# Autodesk Inventor assembly: printer
(part 2 of 3)
532. ISO 4762 M4 x 40:3 — Mate:807, Mate:809, Mate:818, Mate:826
533. ISO 4762 M4 x 40:4 — Mate:808, Mate:812, Mate:820, Mate:824
534. DIN EN ISO 7040 M4:88 — Mate:823, Mate:824
535. DIN EN ISO 7040 M4:89 — Mate:825, Mate:826
536. DIN EN ISO 7040 M4:90 — Mate:827, Mate:828
537. DIN EN ISO 7040 M4:91 — Mate:821, Mate:822
538. CSN 02 1702 B B 4,3:175 — Mate:813, Mate:818, Mate:825
539. CSN 02 1702 B B 4,3:176 — Mate:814, Mate:817, Mate:821
540. CSN 02 1702 B B 4,3:177 — Mate:815, Mate:820, Mate:823
541. CSN 02 1702 B B 4,3:178 — Mate:816, Mate:819, Mate:827
## Relationships (1028: Mate 807, Insert 155, Angle 45, Flush 17, Tangent 4)
- Mate:1: brace_left:1
- Mate:2: brace_left:1
- Flush:1: brace_left:1
- Mate:3: brace_left:1 ↔ frame:1
- Mate:4: brace_left:1 ↔ frame:1
- Mate:5: brace_left:1 ↔ frame:1
- Mate:6: frame:1 ↔ z_motor_mount:1
- Flush:2: frame:1 ↔ z_motor_mount:1
- Flush:3: frame:1 ↔ z_motor_mount:1
- Mate:7: frame:1 ↔ z_motor_mount:2
- Flush:4: frame:1 ↔ z_motor_mount:2
- Flush:5: frame:1 ↔ z_motor_mount:2
- Mate:8: z_motor_mount:1 ↔ z_rod_stopper_bottom:1
- Mate:9: z_motor_mount:1 ↔ z_rod_stopper_bottom:1
- Mate:10: z_motor_mount:1 ↔ z_rod_stopper_bottom:1
- Mate:11: z_motor_mount:2 ↔ z_rod_stopper_bottom:2
- Mate:12: z_motor_mount:2 ↔ z_rod_stopper_bottom:2
- Mate:13: z_motor_mount:2 ↔ z_rod_stopper_bottom:2
- Mate:14: z_motor_mount:1 ↔ CSN 02 1702 B B 4,3:5
- Mate:15: z_motor_mount:1 ↔ CSN 02 1702 B B 4,3:6
- Mate:16: z_motor_mount:1 ↔ CSN 02 1702 B B 4,3:5
- Mate:17: z_motor_mount:1 ↔ CSN 02 1702 B B 4,3:6
- Insert:1: CSN 02 1702 B B 4,3:5 ↔ ISO 4762 M4 x 20:4
- Insert:2: CSN 02 1702 B B 4,3:6 ↔ ISO 4762 M4 x 20:3
- Mate:18: z_rod_stopper_bottom:1 ↔ CSN 02 1702 B B 4,3:3
- Mate:19: CSN 02 1702 B B 4,3:3 ↔ ISO 4762 M4 x 20:3
- Mate:20: z_rod_stopper_bottom:1 ↔ CSN 02 1702 B B 4,3:4
- Mate:21: CSN 02 1702 B B 4,3:4 ↔ ISO 4762 M4 x 20:4
- Mate:22: z_motor_mount:2 ↔ CSN 02 1702 B B 4,3:1
- Mate:23: z_motor_mount:2 ↔ CSN 02 1702 B B 4,3:1
- Mate:24: z_motor_mount:2 ↔ CSN 02 1702 B B 4,3:8
- Mate:25: z_motor_mount:2 ↔ CSN 02 1702 B B 4,3:8
- Insert:3: CSN 02 1702 B B 4,3:8 ↔ ISO 4762 M4 x 20:2
- Insert:4: CSN 02 1702 B B 4,3:1 ↔ ISO 4762 M4 x 20:1
- Mate:26: z_rod_stopper_bottom:2 ↔ CSN 02 1702 B B 4,3:2
- Mate:27: CSN 02 1702 B B 4,3:2 ↔ ISO 4762 M4 x 20:2
- Mate:28: z_rod_stopper_bottom:2 ↔ CSN 02 1702 B B 4,3:7
- Mate:29: CSN 02 1702 B B 4,3:7 ↔ ISO 4762 M4 x 20:1
- Mate:30: CSN 02 1702 B B 4,3:3 ↔ DIN EN ISO 7040 M4:4
- Mate:31: ISO 4762 M4 x 20:3 ↔ DIN EN ISO 7040 M4:4
- Mate:32: CSN 02 1702 B B 4,3:4 ↔ DIN EN ISO 7040 M4:3
- Mate:33: ISO 4762 M4 x 20:4 ↔ DIN EN ISO 7040 M4:3
- Mate:34: CSN 02 1702 B B 4,3:2 ↔ DIN EN ISO 7040 M4:2
- Mate:35: ISO 4762 M4 x 20:2 ↔ DIN EN ISO 7040 M4:2
- Mate:36: CSN 02 1702 B B 4,3:7 ↔ DIN EN ISO 7040 M4:1
- Mate:37: ISO 4762 M4 x 20:1 ↔ DIN EN ISO 7040 M4:1
- Mate:38: z_rod_stopper_bottom:1 ↔ NEMA 17:1
- Mate:39: z_rod_stopper_bottom:1 ↔ NEMA 17:1
- Mate:40: z_rod_stopper_bottom:1 ↔ NEMA 17:1
- Mate:41: z_rod_stopper_bottom:2 ↔ NEMA 17:2
- Mate:42: z_rod_stopper_bottom:2 ↔ NEMA 17:2
- Mate:43: z_rod_stopper_bottom:2 ↔ NEMA 17:2
- Mate:44: z_motor_mount:1 ↔ CSN 02 1702 B B 3,2:8
- Mate:45: z_motor_mount:1 ↔ CSN 02 1702 B B 3,2:1
- Mate:46: z_motor_mount:1 ↔ CSN 02 1702 B B 3,2:6
- Mate:47: z_motor_mount:1 ↔ CSN 02 1702 B B 3,2:7
- Mate:48: z_motor_mount:2 ↔ CSN 02 1702 B B 3,2:2
- Mate:49: z_motor_mount:2 ↔ CSN 02 1702 B B 3,2:3
- Mate:50: z_motor_mount:2 ↔ CSN 02 1702 B B 3,2:4
- Mate:51: z_motor_mount:2 ↔ CSN 02 1702 B B 3,2:5
- Mate:52: z_motor_mount:1 ↔ CSN 02 1702 B B 3,2:8
- Mate:53: z_motor_mount:1 ↔ CSN 02 1702 B B 3,2:1
- Mate:54: z_motor_mount:1 ↔ CSN 02 1702 B B 3,2:7
- Mate:55: z_motor_mount:1 ↔ CSN 02 1702 B B 3,2:6
- Mate:56: z_motor_mount:2 ↔ CSN 02 1702 B B 3,2:5
- Mate:57: z_motor_mount:2 ↔ CSN 02 1702 B B 3,2:2
- Mate:58: z_motor_mount:2 ↔ CSN 02 1702 B B 3,2:4
- Mate:59: z_motor_mount:2 ↔ CSN 02 1702 B B 3,2:3
- Insert:5: CSN 02 1702 B B 3,2:7 ↔ ISO 4762 M3 x 20:8
- Insert:6: CSN 02 1702 B B 3,2:8 ↔ ISO 4762 M3 x 20:7
- Insert:7: CSN 02 1702 B B 3,2:6 ↔ ISO 4762 M3 x 20:6
- Insert:8: CSN 02 1702 B B 3,2:1 ↔ ISO 4762 M3 x 20:5
- Insert:9: CSN 02 1702 B B 3,2:5 ↔ ISO 4762 M3 x 20:4
- Insert:10: CSN 02 1702 B B 3,2:2 ↔ ISO 4762 M3 x 20:3
- Insert:11: CSN 02 1702 B B 3,2:3 ↔ ISO 4762 M3 x 20:2
- Insert:12: CSN 02 1702 B B 3,2:4 ↔ ISO 4762 M3 x 20:1
- Insert:13: z_motor_mount:1 ↔ z_axis_rod:2
- Insert:14: z_motor_mount:2 ↔ z_axis_rod:1
- Mate:60: z_motor_mount:2 ↔ z_motor_brace:1
- Mate:61: z_motor_mount:2 ↔ z_motor_brace:1
- Mate:62: z_motor_mount:2 ↔ z_motor_brace:1
- Mate:63: z_motor_mount:1 ↔ z_motor_brace:2
- Mate:64: z_motor_mount:1 ↔ z_motor_brace:2
- Mate:65: z_motor_mount:1 ↔ z_motor_brace:2
- Mate:66: NEMA 17:1 ↔ z_threaded_rod:1
- Mate:67: NEMA 17:1 ↔ z_threaded_rod:1
- Mate:68: NEMA 17:2 ↔ z_threaded_rod:2
- Mate:69: NEMA 17:2 ↔ z_threaded_rod:2
- Mate:70: frame:1 ↔ frame_brace_top:1
- Mate:71: brace_left:1 ↔ frame_brace_top:1
- Mate:72: frame:1 ↔ frame_brace_top:1
- Mate:73: brace_left:1 ↔ front:1
- Flush:6: brace_left:1 ↔ front:1
- Flush:7 (-3 mm): brace_left:1 ↔ front:1
- Mate:74: frame:1 ↔ z_axis_top:1
- Mate:75: frame:1 ↔ z_axis_top:1
- Mate:76: frame:1 ↔ z_axis_top:1
- Mate:77: frame:1 ↔ z_axis_top:2
- Mate:78: frame:1 ↔ z_axis_top:2
- Mate:79: frame:1 ↔ z_axis_top:2
- Mate:80: brace_left:1 ↔ bottom:1
- Mate:81: front:1 ↔ bottom:1
- Flush:8 (3 mm): brace_left:1 ↔ bottom:1
- Mate:84: frame:1 ↔ wiring_brace:1
- Flush:9: frame:1 ↔ wiring_brace:1
- Mate:85: brace_left:1 ↔ wiring_brace:1
- Mate:86: frame:1 ↔ wiring_brace:2
- Flush:10: frame:1 ↔ wiring_brace:2
- Mate:87: frame:1 ↔ wiring_brace:2
- Mate:88: frame:1 ↔ brace_right:1
- Mate:89: bottom:1 ↔ brace_right:1
- Flush:11 (-3 mm): bottom:1 ↔ brace_right:1
- Mate:90: brace_right:1 ↔ back:1
- Flush:12 (-3 mm): brace_right:1 ↔ back:1
- Flush:13 (-3 mm): bottom:1 ↔ back:1
- Insert:15: front:1 ↔ y_axis_rod:2
- Insert:16: front:1 ↔ y_axis_rod:1
- Mate:91: front:1 ↔ CSN 02 1702 B B 4,3:18
- Mate:92: front:1 ↔ CSN 02 1702 B B 4,3:17
- Mate:93: front:1 ↔ CSN 02 1702 B B 4,3:16
- Mate:94: front:1 ↔ CSN 02 1702 B B 4,3:13
- Mate:95: front:1 ↔ CSN 02 1702 B B 4,3:14
- Mate:96: front:1 ↔ CSN 02 1702 B B 4,3:15
- Mate:97: front:1 ↔ CSN 02 1702 B B 4,3:9
- Mate:98: front:1 ↔ CSN 02 1702 B B 4,3:10
- Mate:99: front:1 ↔ CSN 02 1702 B B 4,3:11
- Mate:100: front:1 ↔ CSN 02 1702 B B 4,3:22
- Mate:101: front:1 ↔ CSN 02 1702 B B 4,3:18
- Mate:102: front:1 ↔ CSN 02 1702 B B 4,3:17
- Mate:103: front:1 ↔ CSN 02 1702 B B 4,3:16
- Mate:104: front:1 ↔ CSN 02 1702 B B 4,3:13
- Mate:105: front:1 ↔ CSN 02 1702 B B 4,3:14
- Mate:106: front:1 ↔ CSN 02 1702 B B 4,3:15
- Mate:107: front:1 ↔ CSN 02 1702 B B 4,3:9
- Mate:108: front:1 ↔ CSN 02 1702 B B 4,3:10
- Mate:109: front:1 ↔ CSN 02 1702 B B 4,3:11
- Mate:110: front:1 ↔ CSN 02 1702 B B 4,3:22
- Insert:17: CSN 02 1702 B B 4,3:18 ↔ ISO 4762 M4 x 20:5
- Insert:18: CSN 02 1702 B B 4,3:17 ↔ ISO 4762 M4 x 20:6
- Insert:19: CSN 02 1702 B B 4,3:16 ↔ ISO 4762 M4 x 20:7
- Insert:20: CSN 02 1702 B B 4,3:13 ↔ ISO 4762 M4 x 20:8
- Insert:21: CSN 02 1702 B B 4,3:14 ↔ ISO 4762 M4 x 20:9
- Insert:22: CSN 02 1702 B B 4,3:15 ↔ ISO 4762 M4 x 20:10
- Insert:23: CSN 02 1702 B B 4,3:9 ↔ ISO 4762 M4 x 20:11
- Insert:24: CSN 02 1702 B B 4,3:10 ↔ ISO 4762 M4 x 20:12
- Insert:25: CSN 02 1702 B B 4,3:11 ↔ ISO 4762 M4 x 20:13
- Insert:26: CSN 02 1702 B B 4,3:22 ↔ ISO 4762 M4 x 20:14
- Mate:111: brace_left:1 ↔ CSN 02 1702 B B 4,3:28
- Mate:112: CSN 02 1702 B B 4,3:28 ↔ ISO 4762 M4 x 20:5
- Mate:113: brace_left:1 ↔ CSN 02 1702 B B 4,3:25
- Mate:114: CSN 02 1702 B B 4,3:25 ↔ ISO 4762 M4 x 20:6
- Mate:115: brace_left:1 ↔ CSN 02 1702 B B 4,3:21
- Mate:116: CSN 02 1702 B B 4,3:21 ↔ ISO 4762 M4 x 20:7
- Mate:117: bottom:1 ↔ CSN 02 1702 B B 4,3:20
- Mate:118: CSN 02 1702 B B 4,3:20 ↔ ISO 4762 M4 x 20:8
- Mate:119: bottom:1 ↔ CSN 02 1702 B B 4,3:27
- Mate:120: CSN 02 1702 B B 4,3:27 ↔ ISO 4762 M4 x 20:9
- Mate:121: bottom:1 ↔ CSN 02 1702 B B 4,3:24
- Mate:122: CSN 02 1702 B B 4,3:24 ↔ ISO 4762 M4 x 20:10
- Mate:123: bottom:1 ↔ CSN 02 1702 B B 4,3:26
- Mate:124: CSN 02 1702 B B 4,3:26 ↔ ISO 4762 M4 x 20:11
- Mate:125: brace_right:1 ↔ CSN 02 1702 B B 4,3:23
- Mate:126: CSN 02 1702 B B 4,3:23 ↔ ISO 4762 M4 x 20:14
- Mate:127: brace_right:1 ↔ CSN 02 1702 B B 4,3:19
- Mate:128: CSN 02 1702 B B 4,3:19 ↔ ISO 4762 M4 x 20:13
- Mate:129: brace_right:1 ↔ CSN 02 1702 B B 4,3:12
- Mate:130: CSN 02 1702 B B 4,3:12 ↔ ISO 4762 M4 x 20:12
- Mate:131: CSN 02 1702 B B 4,3:28 ↔ DIN EN ISO 7040 M4:5
- Mate:132: ISO 4762 M4 x 20:5 ↔ DIN EN ISO 7040 M4:5
- Mate:133: CSN 02 1702 B B 4,3:25 ↔ DIN EN ISO 7040 M4:12
- Mate:134: ISO 4762 M4 x 20:6 ↔ DIN EN ISO 7040 M4:12
- Mate:135: CSN 02 1702 B B 4,3:21 ↔ DIN EN ISO 7040 M4:9
- Mate:136: ISO 4762 M4 x 20:7 ↔ DIN EN ISO 7040 M4:9
- Mate:137: CSN 02 1702 B B 4,3:20 ↔ DIN EN ISO 7040 M4:13
- Mate:138: ISO 4762 M4 x 20:8 ↔ DIN EN ISO 7040 M4:13
- Mate:139: CSN 02 1702 B B 4,3:27 ↔ DIN EN ISO 7040 M4:14
- Mate:140: ISO 4762 M4 x 20:9 ↔ DIN EN ISO 7040 M4:14
- Mate:141: CSN 02 1702 B B 4,3:24 ↔ DIN EN ISO 7040 M4:6
- Mate:142: ISO 4762 M4 x 20:10 ↔ DIN EN ISO 7040 M4:6
- Mate:143: CSN 02 1702 B B 4,3:26 ↔ DIN EN ISO 7040 M4:7
- Mate:144: ISO 4762 M4 x 20:11 ↔ DIN EN ISO 7040 M4:7
- Mate:145: CSN 02 1702 B B 4,3:23 ↔ DIN EN ISO 7040 M4:10
- Mate:146: ISO 4762 M4 x 20:14 ↔ DIN EN ISO 7040 M4:10
- Mate:147: CSN 02 1702 B B 4,3:19 ↔ DIN EN ISO 7040 M4:8
- Mate:148: ISO 4762 M4 x 20:13 ↔ DIN EN ISO 7040 M4:8
- Mate:149: CSN 02 1702 B B 4,3:12 ↔ DIN EN ISO 7040 M4:11
- Mate:150: ISO 4762 M4 x 20:12 ↔ DIN EN ISO 7040 M4:11
- Mate:151: back:1 ↔ CSN 02 1702 B B 4,3:29
- Mate:152: back:1 ↔ CSN 02 1702 B B 4,3:30
- Mate:153: back:1 ↔ CSN 02 1702 B B 4,3:32
- Mate:154: back:1 ↔ CSN 02 1702 B B 4,3:33
- Mate:155: back:1 ↔ CSN 02 1702 B B 4,3:35
- Mate:156: back:1 ↔ CSN 02 1702 B B 4,3:36
- Mate:157: back:1 ↔ CSN 02 1702 B B 4,3:37
- Mate:158: back:1 ↔ CSN 02 1702 B B 4,3:38
- Mate:159: back:1 ↔ CSN 02 1702 B B 4,3:34
- Mate:160: back:1 ↔ CSN 02 1702 B B 4,3:31
- Mate:161: back:1 ↔ CSN 02 1702 B B 4,3:31
- Mate:162: back:1 ↔ CSN 02 1702 B B 4,3:34
- Mate:163: back:1 ↔ CSN 02 1702 B B 4,3:38
- Mate:164: back:1 ↔ CSN 02 1702 B B 4,3:37
- Mate:165: back:1 ↔ CSN 02 1702 B B 4,3:36
- Mate:166: back:1 ↔ CSN 02 1702 B B 4,3:35
- Mate:167: back:1 ↔ CSN 02 1702 B B 4,3:33
- Mate:168: back:1 ↔ CSN 02 1702 B B 4,3:29
- Mate:169: back:1 ↔ CSN 02 1702 B B 4,3:30
- Mate:170: back:1 ↔ CSN 02 1702 B B 4,3:32
- Insert:27: CSN 02 1702 B B 4,3:32 ↔ ISO 4762 M4 x 20:15
- Insert:28: CSN 02 1702 B B 4,3:30 ↔ ISO 4762 M4 x 20:16
- Insert:29: CSN 02 1702 B B 4,3:29 ↔ ISO 4762 M4 x 20:17
- Insert:30: CSN 02 1702 B B 4,3:33 ↔ ISO 4762 M4 x 20:18
- Insert:31: CSN 02 1702 B B 4,3:35 ↔ ISO 4762 M4 x 20:19
- Insert:32: CSN 02 1702 B B 4,3:36 ↔ ISO 4762 M4 x 20:20
- Insert:33: CSN 02 1702 B B 4,3:37 ↔ ISO 4762 M4 x 20:21
- Insert:34: CSN 02 1702 B B 4,3:38 ↔ ISO 4762 M4 x 20:22
- Insert:35: CSN 02 1702 B B 4,3:34 ↔ ISO 4762 M4 x 20:23
- Insert:36: CSN 02 1702 B B 4,3:31 ↔ ISO 4762 M4 x 20:24
- Mate:171: brace_right:1 ↔ CSN 02 1702 B B 4,3:39
- Mate:172: CSN 02 1702 B B 4,3:39 ↔ ISO 4762 M4 x 20:24
- Mate:173: brace_right:1 ↔ CSN 02 1702 B B 4,3:41
- Mate:174: CSN 02 1702 B B 4,3:41 ↔ ISO 4762 M4 x 20:23
- Mate:175: brace_right:1 ↔ CSN 02 1702 B B 4,3:40
- Mate:176: CSN 02 1702 B B 4,3:40 ↔ ISO 4762 M4 x 20:22
- Mate:177: brace_left:1 ↔ CSN 02 1702 B B 4,3:42
- Mate:178: CSN 02 1702 B B 4,3:42 ↔ ISO 4762 M4 x 20:15
- Mate:179: brace_left:1 ↔ CSN 02 1702 B B 4,3:45
- Mate:180: CSN 02 1702 B B 4,3:45 ↔ ISO 4762 M4 x 20:16
- Mate:181: brace_left:1 ↔ CSN 02 1702 B B 4,3:43
- Mate:182: CSN 02 1702 B B 4,3:43 ↔ ISO 4762 M4 x 20:17
- Mate:183: bottom:1 ↔ CSN 02 1702 B B 4,3:46
- Mate:184: CSN 02 1702 B B 4,3:46 ↔ ISO 4762 M4 x 20:18
- Mate:185: bottom:1 ↔ CSN 02 1702 B B 4,3:47
- Mate:186: CSN 02 1702 B B 4,3:47 ↔ ISO 4762 M4 x 20:19
- Mate:187: bottom:1 ↔ CSN 02 1702 B B 4,3:44
- Mate:188: CSN 02 1702 B B 4,3:44 ↔ ISO 4762 M4 x 20:20
- Mate:189: bottom:1 ↔ CSN 02 1702 B B 4,3:48
- Mate:190: CSN 02 1702 B B 4,3:48 ↔ ISO 4762 M4 x 20:21
- Mate:191: CSN 02 1702 B B 4,3:42 ↔ DIN EN ISO 7040 M4:17
- Mate:192: ISO 4762 M4 x 20:15 ↔ DIN EN ISO 7040 M4:17
- Mate:193: CSN 02 1702 B B 4,3:45 ↔ DIN EN ISO 7040 M4:15
- Mate:194: ISO 4762 M4 x 20:16 ↔ DIN EN ISO 7040 M4:15
- Mate:195: CSN 02 1702 B B 4,3:43 ↔ DIN EN ISO 7040 M4:22
- Mate:196: ISO 4762 M4 x 20:17 ↔ DIN EN ISO 7040 M4:22
- Mate:197: CSN 02 1702 B B 4,3:46 ↔ DIN EN ISO 7040 M4:23
- Mate:198: ISO 4762 M4 x 20:18 ↔ DIN EN ISO 7040 M4:23
- Mate:199: CSN 02 1702 B B 4,3:47 ↔ DIN EN ISO 7040 M4:24
- Mate:200: ISO 4762 M4 x 20:19 ↔ DIN EN ISO 7040 M4:24
- Mate:201: CSN 02 1702 B B 4,3:44 ↔ DIN EN ISO 7040 M4:18
- Mate:202: ISO 4762 M4 x 20:20 ↔ DIN EN ISO 7040 M4:18
- Mate:203: CSN 02 1702 B B 4,3:48 ↔ DIN EN ISO 7040 M4:21
- Mate:204: ISO 4762 M4 x 20:21 ↔ DIN EN ISO 7040 M4:21
- Mate:205: CSN 02 1702 B B 4,3:39 ↔ DIN EN ISO 7040 M4:20
- Mate:206: ISO 4762 M4 x 20:24 ↔ DIN EN ISO 7040 M4:20
- Mate:207: CSN 02 1702 B B 4,3:41 ↔ DIN EN ISO 7040 M4:16
- Mate:208: ISO 4762 M4 x 20:23 ↔ DIN EN ISO 7040 M4:16
- Mate:209: CSN 02 1702 B B 4,3:40 ↔ DIN EN ISO 7040 M4:19
- Mate:210: ISO 4762 M4 x 20:22 ↔ DIN EN ISO 7040 M4:19
- Mate:211: frame:1 ↔ CSN 02 1702 B B 4,3:49
- Mate:212: frame:1 ↔ CSN 02 1702 B B 4,3:59
- Mate:213: frame:1 ↔ CSN 02 1702 B B 4,3:50
- Mate:214: frame:1 ↔ CSN 02 1702 B B 4,3:51
- Mate:215: frame:1 ↔ CSN 02 1702 B B 4,3:52
- Mate:216: frame:1 ↔ CSN 02 1702 B B 4,3:53
- Mate:217: frame:1 ↔ CSN 02 1702 B B 4,3:54
- Mate:218: frame:1 ↔ CSN 02 1702 B B 4,3:55
- Mate:219: frame:1 ↔ CSN 02 1702 B B 4,3:56
- Mate:220: frame:1 ↔ CSN 02 1702 B B 4,3:57
- Mate:221: frame:1 ↔ CSN 02 1702 B B 4,3:53
- Mate:222: frame:1 ↔ CSN 02 1702 B B 4,3:54
- Mate:223: frame:1 ↔ CSN 02 1702 B B 4,3:55
- Mate:224: frame:1 ↔ CSN 02 1702 B B 4,3:56
- Mate:225: frame:1 ↔ CSN 02 1702 B B 4,3:57
- Mate:226: frame:1 ↔ CSN 02 1702 B B 4,3:49
- Mate:227: frame:1 ↔ CSN 02 1702 B B 4,3:59
- Mate:228: frame:1 ↔ CSN 02 1702 B B 4,3:50
- Mate:229: frame:1 ↔ CSN 02 1702 B B 4,3:51
- Mate:230: frame:1 ↔ CSN 02 1702 B B 4,3:52
- Insert:37: CSN 02 1702 B B 4,3:49 ↔ ISO 4762 M4 x 20:25
- Insert:38: CSN 02 1702 B B 4,3:59 ↔ ISO 4762 M4 x 20:26
- Insert:39: CSN 02 1702 B B 4,3:50 ↔ ISO 4762 M4 x 20:27
- Insert:40: CSN 02 1702 B B 4,3:51 ↔ ISO 4762 M4 x 20:28
- Insert:41: CSN 02 1702 B B 4,3:52 ↔ ISO 4762 M4 x 20:29
- Insert:42: CSN 02 1702 B B 4,3:53 ↔ ISO 4762 M4 x 20:30
- Insert:43: CSN 02 1702 B B 4,3:54 ↔ ISO 4762 M4 x 20:31
- Insert:44: CSN 02 1702 B B 4,3:55 ↔ ISO 4762 M4 x 20:32
- Insert:45: CSN 02 1702 B B 4,3:56 ↔ ISO 4762 M4 x 20:33
- Insert:46: CSN 02 1702 B B 4,3:57 ↔ ISO 4762 M4 x 20:34
- Mate:231: brace_right:1 ↔ CSN 02 1702 B B 4,3:60
- Mate:232: CSN 02 1702 B B 4,3:60 ↔ ISO 4762 M4 x 20:25
- Mate:233: brace_right:1 ↔ CSN 02 1702 B B 4,3:61
- Mate:234: CSN 02 1702 B B 4,3:61 ↔ ISO 4762 M4 x 20:26
- Mate:235: brace_right:1 ↔ CSN 02 1702 B B 4,3:62
- Mate:236: CSN 02 1702 B B 4,3:62 ↔ ISO 4762 M4 x 20:27
- Mate:237: brace_right:1 ↔ CSN 02 1702 B B 4,3:63
- Mate:238: CSN 02 1702 B B 4,3:63 ↔ ISO 4762 M4 x 20:28
- Mate:239: brace_right:1 ↔ CSN 02 1702 B B 4,3:64
- Mate:240: CSN 02 1702 B B 4,3:64 ↔ ISO 4762 M4 x 20:29
- Mate:241: brace_left:1 ↔ CSN 02 1702 B B 4,3:65
- Mate:242: CSN 02 1702 B B 4,3:65 ↔ ISO 4762 M4 x 20:30
- Mate:243: brace_left:1 ↔ CSN 02 1702 B B 4,3:66
- Mate:244: CSN 02 1702 B B 4,3:66 ↔ ISO 4762 M4 x 20:31
- Mate:245: brace_left:1 ↔ CSN 02 1702 B B 4,3:67
- Mate:246: CSN 02 1702 B B 4,3:67 ↔ ISO 4762 M4 x 20:32
- Mate:247: brace_left:1 ↔ CSN 02 1702 B B 4,3:58
- Mate:248: CSN 02 1702 B B 4,3:58 ↔ ISO 4762 M4 x 20:33
- Mate:249: brace_left:1 ↔ CSN 02 1702 B B 4,3:68
- Mate:250: CSN 02 1702 B B 4,3:68 ↔ ISO 4762 M4 x 20:34
- Mate:251: CSN 02 1702 B B 4,3:60 ↔ DIN EN ISO 7040 M4:25
- Mate:252: ISO 4762 M4 x 20:25 ↔ DIN EN ISO 7040 M4:25
- Mate:253: CSN 02 1702 B B 4,3:61 ↔ DIN EN ISO 7040 M4:26
- Mate:254: ISO 4762 M4 x 20:26 ↔ DIN EN ISO 7040 M4:26
- Mate:255: CSN 02 1702 B B 4,3:62 ↔ DIN EN ISO 7040 M4:27
- Mate:256: ISO 4762 M4 x 20:27 ↔ DIN EN ISO 7040 M4:27
- Mate:257: CSN 02 1702 B B 4,3:63 ↔ DIN EN ISO 7040 M4:34
- Mate:258: ISO 4762 M4 x 20:28 ↔ DIN EN ISO 7040 M4:34
- Mate:259: CSN 02 1702 B B 4,3:64 ↔ DIN EN ISO 7040 M4:33
- Mate:260: ISO 4762 M4 x 20:29 ↔ DIN EN ISO 7040 M4:33
- Mate:261: CSN 02 1702 B B 4,3:65 ↔ DIN EN ISO 7040 M4:28
- Mate:262: ISO 4762 M4 x 20:30 ↔ DIN EN ISO 7040 M4:28
- Mate:263: CSN 02 1702 B B 4,3:66 ↔ DIN EN ISO 7040 M4:29
- Mate:264: ISO 4762 M4 x 20:31 ↔ DIN EN ISO 7040 M4:29
- Mate:265: CSN 02 1702 B B 4,3:67 ↔ DIN EN ISO 7040 M4:32
- Mate:266: ISO 4762 M4 x 20:32 ↔ DIN EN ISO 7040 M4:32
- Mate:267: CSN 02 1702 B B 4,3:58 ↔ DIN EN ISO 7040 M4:30
- Mate:268: ISO 4762 M4 x 20:33 ↔ DIN EN ISO 7040 M4:30
- Mate:269: CSN 02 1702 B B 4,3:68 ↔ DIN EN ISO 7040 M4:31
- Mate:270: ISO 4762 M4 x 20:34 ↔ DIN EN ISO 7040 M4:31
- Mate:271: brace_right:1 ↔ CSN 02 1702 B B 4,3:69
- Mate:272: brace_right:1 ↔ CSN 02 1702 B B 4,3:70
- Mate:273: brace_right:1 ↔ CSN 02 1702 B B 4,3:71
- Mate:274: brace_right:1 ↔ CSN 02 1702 B B 4,3:72
- Mate:275: brace_right:1 ↔ CSN 02 1702 B B 4,3:73
- Mate:276: brace_left:1 ↔ CSN 02 1702 B B 4,3:74
- Mate:277: brace_left:1 ↔ CSN 02 1702 B B 4,3:75
- Mate:278: brace_left:1 ↔ CSN 02 1702 B B 4,3:76
- Mate:279: brace_left:1 ↔ CSN 02 1702 B B 4,3:77
- Mate:280: brace_left:1 ↔ CSN 02 1702 B B 4,3:78
- Mate:281: brace_left:1 ↔ CSN 02 1702 B B 4,3:74
- Mate:282: brace_left:1 ↔ CSN 02 1702 B B 4,3:75
- Mate:283: brace_left:1 ↔ CSN 02 1702 B B 4,3:76
- Mate:284: brace_left:1 ↔ CSN 02 1702 B B 4,3:77
- Mate:285: brace_left:1 ↔ CSN 02 1702 B B 4,3:78
- Mate:286: brace_right:1 ↔ CSN 02 1702 B B 4,3:73
- Mate:287: brace_right:1 ↔ CSN 02 1702 B B 4,3:72
- Mate:288: brace_right:1 ↔ CSN 02 1702 B B 4,3:71
- Mate:289: brace_right:1 ↔ CSN 02 1702 B B 4,3:70
- Mate:290: brace_right:1 ↔ CSN 02 1702 B B 4,3:69
- Insert:47: CSN 02 1702 B B 4,3:73 ↔ ISO 4762 M4 x 20:44
- Insert:48: CSN 02 1702 B B 4,3:72 ↔ ISO 4762 M4 x 20:43
- Insert:49: CSN 02 1702 B B 4,3:71 ↔ ISO 4762 M4 x 20:42
- Insert:50: CSN 02 1702 B B 4,3:70 ↔ ISO 4762 M4 x 20:41
- Insert:51: CSN 02 1702 B B 4,3:69 ↔ ISO 4762 M4 x 20:40
- Insert:52: CSN 02 1702 B B 4,3:78 ↔ ISO 4762 M4 x 20:39
- Insert:53: CSN 02 1702 B B 4,3:77 ↔ ISO 4762 M4 x 20:38
- Insert:54: CSN 02 1702 B B 4,3:76 ↔ ISO 4762 M4 x 20:37
- Insert:55: CSN 02 1702 B B 4,3:75 ↔ ISO 4762 M4 x 20:36
- Insert:56: CSN 02 1702 B B 4,3:74 ↔ ISO 4762 M4 x 20:35
- Mate:291: bottom:1 ↔ CSN 02 1702 B B 4,3:88
- Mate:292: CSN 02 1702 B B 4,3:88 ↔ ISO 4762 M4 x 20:39
- Mate:293: bottom:1 ↔ CSN 02 1702 B B 4,3:87
- Mate:294: CSN 02 1702 B B 4,3:87 ↔ ISO 4762 M4 x 20:38
- Mate:295: bottom:1 ↔ CSN 02 1702 B B 4,3:86
- Mate:296: CSN 02 1702 B B 4,3:86 ↔ ISO 4762 M4 x 20:37
- Mate:297: bottom:1 ↔ CSN 02 1702 B B 4,3:85
- Mate:298: CSN 02 1702 B B 4,3:85 ↔ ISO 4762 M4 x 20:36
- Mate:299: bottom:1 ↔ CSN 02 1702 B B 4,3:84
- Mate:300: CSN 02 1702 B B 4,3:84 ↔ ISO 4762 M4 x 20:35
- Mate:301: bottom:1 ↔ CSN 02 1702 B B 4,3:83
- Mate:302: CSN 02 1702 B B 4,3:83 ↔ ISO 4762 M4 x 20:40
- Mate:303: bottom:1 ↔ CSN 02 1702 B B 4,3:79
- Mate:304: CSN 02 1702 B B 4,3:79 ↔ ISO 4762 M4 x 20:41
- Mate:305: bottom:1 ↔ CSN 02 1702 B B 4,3:80
- Mate:306: CSN 02 1702 B B 4,3:80 ↔ ISO 4762 M4 x 20:42
- Mate:307: bottom:1 ↔ CSN 02 1702 B B 4,3:81
- Mate:308: CSN 02 1702 B B 4,3:81 ↔ ISO 4762 M4 x 20:43
- Mate:309: bottom:1 ↔ CSN 02 1702 B B 4,3:82
- Mate:310: CSN 02 1702 B B 4,3:82 ↔ ISO 4762 M4 x 20:44
- Mate:311: CSN 02 1702 B B 4,3:82 ↔ DIN EN ISO 7040 M4:41
- Mate:312: ISO 4762 M4 x 20:44 ↔ DIN EN ISO 7040 M4:41
- Mate:313: CSN 02 1702 B B 4,3:81 ↔ DIN EN ISO 7040 M4:40
- Mate:314: ISO 4762 M4 x 20:43 ↔ DIN EN ISO 7040 M4:40
- Mate:315: CSN 02 1702 B B 4,3:80 ↔ DIN EN ISO 7040 M4:39
- Mate:316: ISO 4762 M4 x 20:42 ↔ DIN EN ISO 7040 M4:39
- Mate:317: CSN 02 1702 B B 4,3:79 ↔ DIN EN ISO 7040 M4:38
- Mate:318: ISO 4762 M4 x 20:41 ↔ DIN EN ISO 7040 M4:38
- Mate:319: CSN 02 1702 B B 4,3:83 ↔ DIN EN ISO 7040 M4:42
- Mate:320: ISO 4762 M4 x 20:40 ↔ DIN EN ISO 7040 M4:42
- Mate:321: CSN 02 1702 B B 4,3:88 ↔ DIN EN ISO 7040 M4:37
- Mate:322: ISO 4762 M4 x 20:39 ↔ DIN EN ISO 7040 M4:37
- Mate:323: CSN 02 1702 B B 4,3:87 ↔ DIN EN ISO 7040 M4:43
- Mate:324: ISO 4762 M4 x 20:38 ↔ DIN EN ISO 7040 M4:43
- Mate:325: CSN 02 1702 B B 4,3:85 ↔ DIN EN ISO 7040 M4:44
- Mate:326: ISO 4762 M4 x 20:36 ↔ DIN EN ISO 7040 M4:44
- Mate:327: CSN 02 1702 B B 4,3:86 ↔ DIN EN ISO 7040 M4:36
- Mate:328: ISO 4762 M4 x 20:37 ↔ DIN EN ISO 7040 M4:36
- Mate:329: CSN 02 1702 B B 4,3:84 ↔ DIN EN ISO 7040 M4:35
- Mate:330: ISO 4762 M4 x 20:35 ↔ DIN EN ISO 7040 M4:35
- Mate:331: z_motor_mount:2 ↔ CSN 02 1702 B B 4,3:98
- Mate:332: z_motor_mount:2 ↔ CSN 02 1702 B B 4,3:97
- Mate:333: frame:1 ↔ CSN 02 1702 B B 4,3:96
- Mate:334: frame:1 ↔ CSN 02 1702 B B 4,3:95
- Mate:335: frame:1 ↔ CSN 02 1702 B B 4,3:94
- Mate:336: frame:1 ↔ CSN 02 1702 B B 4,3:93
- Mate:337: frame:1 ↔ CSN 02 1702 B B 4,3:92
- Mate:338: frame:1 ↔ CSN 02 1702 B B 4,3:91
- Mate:339: z_motor_mount:1 ↔ CSN 02 1702 B B 4,3:90
- Mate:340: z_motor_mount:1 ↔ CSN 02 1702 B B 4,3:89
- Mate:341: z_motor_mount:1 ↔ CSN 02 1702 B B 4,3:89
- Mate:342: z_motor_mount:1 ↔ CSN 02 1702 B B 4,3:90
- Mate:343: frame:1 ↔ CSN 02 1702 B B 4,3:93
- Mate:344: frame:1 ↔ CSN 02 1702 B B 4,3:92
- Mate:345: frame:1 ↔ CSN 02 1702 B B 4,3:91
- Mate:346: frame:1 ↔ CSN 02 1702 B B 4,3:96
- Mate:347: frame:1 ↔ CSN 02 1702 B B 4,3:95
- Mate:348: frame:1 ↔ CSN 02 1702 B B 4,3:94
- Mate:349: z_motor_mount:2 ↔ CSN 02 1702 B B 4,3:97
- Mate:350: z_motor_mount:2 ↔ CSN 02 1702 B B 4,3:98
- Insert:57: CSN 02 1702 B B 4,3:97 ↔ ISO 4762 M4 x 20:54
- Insert:58: CSN 02 1702 B B 4,3:98 ↔ ISO 4762 M4 x 20:53
- Insert:59: CSN 02 1702 B B 4,3:95 ↔ ISO 4762 M4 x 20:52
- Insert:60: CSN 02 1702 B B 4,3:96 ↔ ISO 4762 M4 x 20:51
- Insert:61: CSN 02 1702 B B 4,3:94 ↔ ISO 4762 M4 x 20:50
- Insert:62: CSN 02 1702 B B 4,3:93 ↔ ISO 4762 M4 x 20:49
- Insert:63: CSN 02 1702 B B 4,3:92 ↔ ISO 4762 M4 x 20:48
- Insert:64: CSN 02 1702 B B 4,3:91 ↔ ISO 4762 M4 x 20:45
- Insert:65: CSN 02 1702 B B 4,3:89 ↔ ISO 4762 M4 x 20:46
- Insert:66: CSN 02 1702 B B 4,3:90 ↔ ISO 4762 M4 x 20:47
- Mate:351: z_motor_brace:1 ↔ CSN 02 1702 B B 4,3:108
- Mate:352: CSN 02 1702 B B 4,3:108 ↔ ISO 4762 M4 x 20:54
- Mate:353: brace_right:1 ↔ CSN 02 1702 B B 4,3:107
- Mate:354: CSN 02 1702 B B 4,3:107 ↔ ISO 4762 M4 x 20:53
- Mate:355: z_motor_mount:2 ↔ CSN 02 1702 B B 4,3:106
- Mate:356: CSN 02 1702 B B 4,3:106 ↔ ISO 4762 M4 x 20:52
- Mate:357: z_motor_mount:2 ↔ CSN 02 1702 B B 4,3:105
- Mate:358: CSN 02 1702 B B 4,3:105 ↔ ISO 4762 M4 x 20:51
- Mate:359: z_motor_mount:1 ↔ CSN 02 1702 B B 4,3:104
- Mate:360: CSN 02 1702 B B 4,3:104 ↔ ISO 4762 M4 x 20:48
- Mate:361: z_motor_mount:1 ↔ CSN 02 1702 B B 4,3:103
- Mate:362: CSN 02 1702 B B 4,3:103 ↔ ISO 4762 M4 x 20:49
- Mate:363: z_motor_brace:2 ↔ CSN 02 1702 B B 4,3:102
- Mate:364: CSN 02 1702 B B 4,3:102 ↔ ISO 4762 M4 x 20:45
- Mate:365: z_motor_brace:2 ↔ CSN 02 1702 B B 4,3:101
- Mate:366: CSN 02 1702 B B 4,3:101 ↔ ISO 4762 M4 x 20:46
- Mate:367: brace_left:1 ↔ CSN 02 1702 B B 4,3:99
- Mate:368: CSN 02 1702 B B 4,3:99 ↔ ISO 4762 M4 x 20:47
- Mate:369: z_motor_brace:1 ↔ CSN 02 1702 B B 4,3:100
- Mate:370: CSN 02 1702 B B 4,3:100 ↔ ISO 4762 M4 x 20:50
- Mate:371: CSN 02 1702 B B 4,3:106 ↔ DIN EN ISO 7040 M4:54
- Mate:372: ISO 4762 M4 x 20:52 ↔ DIN EN ISO 7040 M4:54
- Mate:373: CSN 02 1702 B B 4,3:105 ↔ DIN EN ISO 7040 M4:52
- Mate:374: ISO 4762 M4 x 20:51 ↔ DIN EN ISO 7040 M4:52
- Mate:375: CSN 02 1702 B B 4,3:100 ↔ DIN EN ISO 7040 M4:53
- Mate:376: ISO 4762 M4 x 20:50 ↔ DIN EN ISO 7040 M4:53
- Mate:377: CSN 02 1702 B B 4,3:108 ↔ DIN EN ISO 7040 M4:51
- Mate:378: ISO 4762 M4 x 20:54 ↔ DIN EN ISO 7040 M4:51
- Mate:379: CSN 02 1702 B B 4,3:107 ↔ DIN EN ISO 7040 M4:50
- Mate:380: ISO 4762 M4 x 20:53 ↔ DIN EN ISO 7040 M4:50
- Mate:381: CSN 02 1702 B B 4,3:102 ↔ DIN EN ISO 7040 M4:49
- Mate:382: ISO 4762 M4 x 20:45 ↔ DIN EN ISO 7040 M4:49
- Mate:383: CSN 02 1702 B B 4,3:101 ↔ DIN EN ISO 7040 M4:48
- Mate:384: ISO 4762 M4 x 20:46 ↔ DIN EN ISO 7040 M4:48
- Mate:385: CSN 02 1702 B B 4,3:99 ↔ DIN EN ISO 7040 M4:47
- Mate:386: ISO 4762 M4 x 20:47 ↔ DIN EN ISO 7040 M4:47
- Mate:387: CSN 02 1702 B B 4,3:104 ↔ DIN EN ISO 7040 M4:46
- Mate:388: ISO 4762 M4 x 20:48 ↔ DIN EN ISO 7040 M4:46
- Mate:389: CSN 02 1702 B B 4,3:103 ↔ DIN EN ISO 7040 M4:45
- Mate:390: ISO 4762 M4 x 20:49 ↔ DIN EN ISO 7040 M4:45
- Mate:391: frame:1 ↔ CSN 02 1702 B B 4,3:120
- Mate:392: brace_right:1 ↔ CSN 02 1702 B B 4,3:115
- Mate:393: brace_right:1 ↔ CSN 02 1702 B B 4,3:109
- Mate:394: brace_right:1 ↔ CSN 02 1702 B B 4,3:109
- Mate:395: brace_left:1 ↔ CSN 02 1702 B B 4,3:114
- Mate:396: brace_left:1 ↔ CSN 02 1702 B B 4,3:114
- Mate:397: frame:1 ↔ CSN 02 1702 B B 4,3:110
- Mate:398: brace_left:1 ↔ CSN 02 1702 B B 4,3:111
- Mate:399: brace_right:1 ↔ CSN 02 1702 B B 4,3:115
- Mate:400: brace_left:1 ↔ CSN 02 1702 B B 4,3:111
- Mate:401: frame:1 ↔ CSN 02 1702 B B 4,3:120
- Mate:402: frame:1 ↔ CSN 02 1702 B B 4,3:110
- Insert:67: CSN 02 1702 B B 4,3:109 ↔ ISO 4762 M4 x 20:60
- Insert:68: CSN 02 1702 B B 4,3:120 ↔ ISO 4762 M4 x 20:59
- Insert:69: CSN 02 1702 B B 4,3:110 ↔ ISO 4762 M4 x 20:58
- Insert:70: CSN 02 1702 B B 4,3:115 ↔ ISO 4762 M4 x 20:57
- Insert:71: CSN 02 1702 B B 4,3:111 ↔ ISO 4762 M4 x 20:56
- Insert:72: CSN 02 1702 B B 4,3:114 ↔ ISO 4762 M4 x 20:55
- Mate:403: frame_brace_top:1 ↔ CSN 02 1702 B B 4,3:113
- Mate:404: CSN 02 1702 B B 4,3:113 ↔ ISO 4762 M4 x 20:55
- Mate:405: frame_brace_top:1 ↔ CSN 02 1702 B B 4,3:116
- Mate:406: CSN 02 1702 B B 4,3:116 ↔ ISO 4762 M4 x 20:60
- Mate:407: wiring_brace:2 ↔ CSN 02 1702 B B 4,3:112
- Mate:408: CSN 02 1702 B B 4,3:112 ↔ ISO 4762 M4 x 20:57
- Mate:409: wiring_brace:1 ↔ CSN 02 1702 B B 4,3:119
- Mate:410: CSN 02 1702 B B 4,3:119 ↔ ISO 4762 M4 x 20:56
- Mate:411: wiring_brace:2 ↔ CSN 02 1702 B B 4,3:117
- Mate:412: CSN 02 1702 B B 4,3:117 ↔ ISO 4762 M4 x 20:59
- Mate:413: wiring_brace:1 ↔ CSN 02 1702 B B 4,3:118
- Mate:414: CSN 02 1702 B B 4,3:118 ↔ ISO 4762 M4 x 20:58
- Mate:415: CSN 02 1702 B B 4,3:112 ↔ DIN EN ISO 7040 M4:60
- Mate:416: ISO 4762 M4 x 20:57 ↔ DIN EN ISO 7040 M4:60
- Mate:417: CSN 02 1702 B B 4,3:117 ↔ DIN EN ISO 7040 M4:59
- Mate:418: ISO 4762 M4 x 20:59 ↔ DIN EN ISO 7040 M4:59
- Mate:419: CSN 02 1702 B B 4,3:116 ↔ DIN EN ISO 7040 M4:58
- Mate:420: ISO 4762 M4 x 20:60 ↔ DIN EN ISO 7040 M4:58
- Mate:421: CSN 02 1702 B B 4,3:118 ↔ DIN EN ISO 7040 M4:57
- Mate:422: ISO 4762 M4 x 20:58 ↔ DIN EN ISO 7040 M4:57
- Mate:423: CSN 02 1702 B B 4,3:119 ↔ DIN EN ISO 7040 M4:56
- Mate:424: ISO 4762 M4 x 20:56 ↔ DIN EN ISO 7040 M4:56
- Mate:425: CSN 02 1702 B B 4,3:113 ↔ DIN EN ISO 7040 M4:55
- Mate:426: ISO 4762 M4 x 20:55 ↔ DIN EN ISO 7040 M4:55
- Mate:427: brace_left:1 ↔ z_axis_cable_mount_a:1
- Mate:428 (18 mm): frame:1 ↔ z_axis_cable_mount_a:1
- Mate:429 (2 mm): frame_brace_top:1 ↔ z_axis_cable_mount_a:1
- Mate:433: z_axis_rod:2 ↔ x_axis:1
- Mate:434: z_axis_rod:1 ↔ x_axis:1
- [Insert]: cable_chain_22:1 ↔ cable_chain_22:2
- [Angle] (0 deg): cable_chain_22:1 ↔ cable_chain_22:2
- [Insert]: cable_chain_22:2 ↔ cable_chain_22:3
- [Angle] (0 deg): cable_chain_22:2 ↔ cable_chain_22:3
- [Insert]: cable_chain_22:4 ↔ cable_chain_22:5
- [Angle] (0 deg): cable_chain_22:4 ↔ cable_chain_22:5
- [Insert]: cable_chain_22:5 ↔ cable_chain_22:6
- [Angle] (0 deg): cable_chain_22:5 ↔ cable_chain_22:6
- [Insert]: cable_chain_22:3 ↔ cable_chain_22:4
- [Angle] (0 deg): cable_chain_22:3 ↔ cable_chain_22:4
- [Insert]: cable_chain_22:7 ↔ cable_chain_22:8
- [Angle] (0 deg): cable_chain_22:7 ↔ cable_chain_22:8
- [Insert]: cable_chain_22:8 ↔ cable_chain_22:9
- [Angle] (0 deg): cable_chain_22:8 ↔ cable_chain_22:9
- [Insert]: cable_chain_22:10 ↔ cable_chain_22:11
- [Angle] (0 deg): cable_chain_22:10 ↔ cable_chain_22:11
- [Insert]: cable_chain_22:11 ↔ cable_chain_22:12
- [Angle] (0 deg): cable_chain_22:11 ↔ cable_chain_22:12
- [Insert]: cable_chain_22:9 ↔ cable_chain_22:10
- [Angle] (0 deg): cable_chain_22:9 ↔ cable_chain_22:10
- [Insert]: cable_chain_22:6 ↔ cable_chain_22:7
- [Angle] (0 deg): cable_chain_22:6 ↔ cable_chain_22:7
- [Insert]: cable_chain_22:13 ↔ cable_chain_22:14
- [Angle] (0 deg): cable_chain_22:13 ↔ cable_chain_22:14
- [Insert]: cable_chain_22:14 ↔ cable_chain_22:15
- [Angle] (0 deg): cable_chain_22:14 ↔ cable_chain_22:15
- [Insert]: cable_chain_22:16 ↔ cable_chain_22:17
- [Angle] (0 deg): cable_chain_22:16 ↔ cable_chain_22:17
- [Insert]: cable_chain_22:17 ↔ cable_chain_22:18
- [Angle] (0 deg): cable_chain_22:17 ↔ cable_chain_22:18
- [Insert]: cable_chain_22:15 ↔ cable_chain_22:16
- [Angle] (0 deg): cable_chain_22:15 ↔ cable_chain_22:16
- [Insert]: cable_chain_22:19 ↔ cable_chain_22:20
- [Angle] (0 deg): cable_chain_22:19 ↔ cable_chain_22:20
- [Insert]: cable_chain_22:18 ↔ cable_chain_22:19
- [Angle] (0 deg): cable_chain_22:18 ↔ cable_chain_22:19
- [Insert]: cable_chain_22:12 ↔ cable_chain_22:13
- [Angle] (0 deg): cable_chain_22:12 ↔ cable_chain_22:13
- Insert:96: z_axis_cable_mount_a:1 ↔ cable_chain_22:1
- Angle:24 (0 deg): z_axis_cable_mount_a:1 ↔ cable_chain_22:1
- Insert:97: cable_chain_22:20 ↔ z_axis_cable_mount_b:1
- Mate:435: x_axis:1 ↔ z_axis_cable_mount_b:1
- Flush:14: x_axis:1 ↔ z_axis_cable_mount_b:1
- Angle:25 (0 deg): cable_chain_22:20 ↔ z_axis_cable_mount_b:1
- Mate:436: y_carriage:1 ↔ y_axis_cable_mount_b:1
- Mate:437: y_carriage:1 ↔ y_axis_cable_mount_b:1
- Mate:438: y_carriage:1 ↔ y_axis_cable_mount_b:1
- [Insert]: cable_chain_22:22 ↔ cable_chain_22:23
- [Angle] (0 deg): cable_chain_22:22 ↔ cable_chain_22:23
- [Insert]: cable_chain_22:24 ↔ cable_chain_22:25
- [Angle] (0 deg): cable_chain_22:24 ↔ cable_chain_22:25
- [Insert]: cable_chain_22:25 ↔ cable_chain_22:26
- [Angle] (0 deg): cable_chain_22:25 ↔ cable_chain_22:26
- [Insert]: cable_chain_22:23 ↔ cable_chain_22:24
- [Angle] (0 deg): cable_chain_22:23 ↔ cable_chain_22:24
- [Insert]: cable_chain_22:27 ↔ cable_chain_22:28
- [Angle] (0 deg): cable_chain_22:27 ↔ cable_chain_22:28
- [Insert]: cable_chain_22:28 ↔ cable_chain_22:29
- [Angle] (0 deg): cable_chain_22:28 ↔ cable_chain_22:29
- [Insert]: cable_chain_22:30 ↔ cable_chain_22:31
- [Angle] (0 deg): cable_chain_22:30 ↔ cable_chain_22:31
- [Insert]: cable_chain_22:31 ↔ cable_chain_22:32
- [Angle] (0 deg): cable_chain_22:31 ↔ cable_chain_22:32
- [Insert]: cable_chain_22:29 ↔ cable_chain_22:30
- [Angle] (0 deg): cable_chain_22:29 ↔ cable_chain_22:30
- [Insert]: cable_chain_22:26 ↔ cable_chain_22:27
- [Angle] (0 deg): cable_chain_22:26 ↔ cable_chain_22:27
- [Insert]: cable_chain_22:33 ↔ cable_chain_22:34
- [Angle] (0 deg): cable_chain_22:33 ↔ cable_chain_22:34
- [Insert]: cable_chain_22:34 ↔ cable_chain_22:35
- [Angle] (0 deg): cable_chain_22:34 ↔ cable_chain_22:35
- [Insert]: cable_chain_22:36 ↔ cable_chain_22:37
- [Angle] (0 deg): cable_chain_22:36 ↔ cable_chain_22:37
- [Insert]: cable_chain_22:37 ↔ cable_chain_22:38
- [Angle] (0 deg): cable_chain_22:37 ↔ cable_chain_22:38
- [Insert]: cable_chain_22:35 ↔ cable_chain_22:36
- [Angle] (0 deg): cable_chain_22:35 ↔ cable_chain_22:36
- [Insert]: cable_chain_22:39 ↔ cable_chain_22:40
- [Angle] (0 deg): cable_chain_22:39 ↔ cable_chain_22:40
- [Insert]: cable_chain_22:40 ↔ cable_chain_22:41
- [Angle] (0 deg): cable_chain_22:40 ↔ cable_chain_22:41
- [Insert]: cable_chain_22:42 ↔ cable_chain_22:43
- [Angle] (0 deg): cable_chain_22:42 ↔ cable_chain_22:43
- [Insert]: cable_chain_22:43 ↔ cable_chain_22:44
- [Angle] (0 deg): cable_chain_22:43 ↔ cable_chain_22:44
- [Insert]: cable_chain_22:41 ↔ cable_chain_22:42
- [Angle] (0 deg): cable_chain_22:41 ↔ cable_chain_22:42
- [Insert]: cable_chain_22:38 ↔ cable_chain_22:39
- [Angle] (0 deg): cable_chain_22:38 ↔ cable_chain_22:39
- [Insert]: cable_chain_22:32 ↔ cable_chain_22:33
- [Angle] (0 deg): cable_chain_22:32 ↔ cable_chain_22:33
- Insert:121: y_axis_cable_mount_b:1 ↔ cable_chain_22:44
- Mate:440: y_axis_rod:2 ↔ y_carriage:1
- Mate:441: y_axis_rod:1 ↔ y_carriage:1
- Angle:65 (0 deg): y_axis_cable_mount_b:1 ↔ cable_chain_22:44
- Insert:122: cable_chain_22:22 ↔ x_axis_cable_mount_a:1
- Angle:66 (0 deg): cable_chain_22:22 ↔ x_axis_cable_mount_a:1
- Mate:442 (30 mm): back:1 ↔ x_axis_cable_mount_a:1
- Mate:443: bottom:1 ↔ x_axis_cable_mount_a:1
- Mate:444: bottom:1 ↔ cable_chain_22:31
- Mate:445: bottom:1 ↔ MW_switching_25A:1
- Mate:446: brace_right:1 ↔ MW_switching_25A:1
- Mate:447 (110 mm): back:1 ↔ MW_switching_25A:1
- Mate:448: 608RS:1 ↔ belt_guide:1
- Mate:449: 608RS:1 ↔ belt_guide:1
- Mate:450: 608RS:1 ↔ belt_guide:2
- Mate:451: belt_guide:1 ↔ belt_guide:2
- Mate:452: belt_guide:1 ↔ belt_guide:2
- Mate:453: 608RS:1 ↔ CSN 02 1702 B B 8,4:1
- Mate:454: 608RS:1 ↔ CSN 02 1702 B B 8,4:1
- Mate:455: CSN 02 1702 B B 8,4:1 ↔ CSN 02 1702 B B 8,4:2
- Mate:456: CSN 02 1702 B B 8,4:1 ↔ CSN 02 1702 B B 8,4:2
- Mate:457: 608RS:1 ↔ CSN 02 1702 B B 8,4:3
- Mate:458: 608RS:1 ↔ CSN 02 1702 B B 8,4:3
- Mate:459: CSN 02 1702 B B 8,4:3 ↔ CSN 02 1702 B B 8,4:4
- Mate:460: CSN 02 1702 B B 8,4:3 ↔ CSN 02 1702 B B 8,4:4
- Mate:461: CSN 02 1702 B B 8,4:2 ↔ y_carriage_belt_iddler:1
- Mate:462: CSN 02 1702 B B 8,4:2 ↔ y_carriage_belt_iddler:1
- Mate:463: y_carriage_belt_iddler:1 ↔ y_carriage_belt_iddler_holder:1
- Mate:464: y_carriage_belt_iddler:1 ↔ y_carriage_belt_iddler_holder:1
- Mate:465: y_carriage_belt_iddler:1 ↔ y_carriage_belt_iddler_holder:1
- Mate:466: y_carriage_belt_iddler:2 ↔ y_carriage_belt_iddler_holder:1
- Mate:467: y_carriage_belt_iddler:2 ↔ y_carriage_belt_iddler_holder:1
- Mate:468: y_carriage_belt_iddler:2 ↔ y_carriage_belt_iddler_holder:1
- Mate:469: back:1 ↔ y_carriage_belt_iddler:2
- Mate:470: y_carriage_belt_iddler:2 ↔ CSN 02 1702 B B 8,4:5
- Mate:471: y_carriage_belt_iddler:2 ↔ CSN 02 1702 B B 8,4:5
- Mate:472: y_carriage_belt_iddler:1 ↔ CSN 02 1702 B B 8,4:6
- Mate:474: CSN 02 1702 B B 8,4:6 ↔ DIN EN ISO 7040 M8:1
- Insert:123: CSN 02 1702 B B 8,4:5 ↔ ISO 4762 M8 x 40:1
- Mate:475: CSN 02 1702 B B 8,4:6 ↔ ISO 4762 M8 x 40:1
- Mate:476: DIN EN ISO 7040 M8:1 ↔ ISO 4762 M8 x 40:1
- Mate:477: back:1 ↔ y_carriage_belt_iddler:2
- Mate:478: back:1 ↔ y_carriage_belt_iddler:2
- Mate:479: back:1 ↔ CSN 02 1702 B B 4,3:124
- Mate:480: back:1 ↔ CSN 02 1702 B B 4,3:123
- Mate:481: back:1 ↔ CSN 02 1702 B B 4,3:123
- Mate:482: back:1 ↔ CSN 02 1702 B B 4,3:124
- Insert:124: CSN 02 1702 B B 4,3:124 ↔ ISO 4762 M4 x 30:1
- Insert:125: CSN 02 1702 B B 4,3:123 ↔ ISO 4762 M4 x 30:2
- Mate:483: y_carriage_belt_iddler_holder:1 ↔ CSN 02 1702 B B 4,3:121
- Mate:484: y_carriage_belt_iddler_holder:1 ↔ CSN 02 1702 B B 4,3:122
- Mate:485: CSN 02 1702 B B 4,3:121 ↔ ISO 4762 M4 x 30:1
- Mate:486: CSN 02 1702 B B 4,3:122 ↔ ISO 4762 M4 x 30:2
- Mate:487: CSN 02 1702 B B 4,3:121 ↔ DIN EN ISO 7040 M4:61
- Mate:488: ISO 4762 M4 x 30:1 ↔ DIN EN ISO 7040 M4:61
- Mate:489: CSN 02 1702 B B 4,3:122 ↔ DIN EN ISO 7040 M4:62
- Mate:490: ISO 4762 M4 x 30:2 ↔ DIN EN ISO 7040 M4:62
- Mate:491: y_motor_mount:1 ↔ y_motor_mount_brace:1
- Mate:492: y_motor_mount:1 ↔ y_motor_mount_brace:1
- Mate:493: y_motor_mount:1 ↔ y_motor_mount_brace:1
- Mate:494: y_motor_mount:1 ↔ motor_spacer:1
- Tangent:1: y_motor_mount:1 ↔ motor_spacer:1
- Tangent:2: y_motor_mount:1 ↔ motor_spacer:1
- Mate:495: front:1 ↔ y_motor_mount:1
- Mate:496: front:1 ↔ y_motor_mount:1
- Mate:497: front:1 ↔ y_motor_mount_brace:1
- Mate:498: front:1 ↔ CSN 02 1702 B B 4,3:127
- Mate:499: front:1 ↔ CSN 02 1702 B B 4,3:128
- Mate:500: front:1 ↔ CSN 02 1702 B B 4,3:128
- Mate:501: front:1 ↔ CSN 02 1702 B B 4,3:127
- Mate:502: y_motor_mount:1 ↔ CSN 02 1702 B B 4,3:130
- Mate:503: y_motor_mount:1 ↔ CSN 02 1702 B B 4,3:130
- Insert:126: CSN 02 1702 B B 4,3:128 ↔ ISO 4762 M4 x 20:61
- Insert:127: CSN 02 1702 B B 4,3:127 ↔ ISO 4762 M4 x 20:62
- Insert:128: CSN 02 1702 B B 4,3:130 ↔ ISO 4762 M4 x 20:63
- Mate:504: y_motor_mount_brace:1 ↔ CSN 02 1702 B B 4,3:125
- Mate:505: y_motor_mount_brace:1 ↔ CSN 02 1702 B B 4,3:129
- Mate:506: CSN 02 1702 B B 4,3:129 ↔ ISO 4762 M4 x 20:62
- Mate:507: CSN 02 1702 B B 4,3:125 ↔ ISO 4762 M4 x 20:63
- Mate:508: y_motor_mount:1 ↔ CSN 02 1702 B B 4,3:126
- Mate:509: CSN 02 1702 B B 4,3:126 ↔ ISO 4762 M4 x 20:61
- Mate:510: CSN 02 1702 B B 4,3:129 ↔ DIN EN ISO 7040 M4:65
- Mate:511: ISO 4762 M4 x 20:62 ↔ DIN EN ISO 7040 M4:65
- Mate:512: CSN 02 1702 B B 4,3:125 ↔ DIN EN ISO 7040 M4:63
- Mate:513: ISO 4762 M4 x 20:63 ↔ DIN EN ISO 7040 M4:63
- Mate:514: CSN 02 1702 B B 4,3:126 ↔ DIN EN ISO 7040 M4:64
- Mate:515: ISO 4762 M4 x 20:61 ↔ DIN EN ISO 7040 M4:64
- Mate:516: motor_spacer:1 ↔ NEMA 17 with T5 Pulley:1
- Mate:517: motor_spacer:1 ↔ NEMA 17 with T5 Pulley:1
- Mate:518: motor_spacer:1 ↔ NEMA 17 with T5 Pulley:1
- Mate:519: y_motor_mount:1 ↔ CSN 02 1702 B B 3,2:9
- Mate:520: y_motor_mount:1 ↔ CSN 02 1702 B B 3,2:10
- Mate:521: y_motor_mount:1 ↔ CSN 02 1702 B B 3,2:11
- Mate:522: y_motor_mount:1 ↔ CSN 02 1702 B B 3,2:12
- Mate:523: motor_spacer:1 ↔ CSN 02 1702 B B 3,2:9
- Mate:524: motor_spacer:1 ↔ CSN 02 1702 B B 3,2:10
- Mate:525: motor_spacer:1 ↔ CSN 02 1702 B B 3,2:11
- Mate:526: motor_spacer:1 ↔ CSN 02 1702 B B 3,2:12
- Insert:129: CSN 02 1702 B B 3,2:10 ↔ ISO 4762 M3 x 20:12
- Insert:130: CSN 02 1702 B B 3,2:9 ↔ ISO 4762 M3 x 20:11
- Insert:131: CSN 02 1702 B B 3,2:12 ↔ ISO 4762 M3 x 20:10
- Insert:132: CSN 02 1702 B B 3,2:11 ↔ ISO 4762 M3 x 20:9
- Mate:527: z_axis_top:1 ↔ rope_mount_a:1
- Flush:15 (3 mm): z_axis_top:1 ↔ rope_mount_a:1
- Mate:528: z_axis_top:1 ↔ rope_mount_a:1
- Mate:529: z_axis_top:1 ↔ rope_mount_b:1
- Flush:16 (3 mm): z_axis_top:1 ↔ rope_mount_b:1
- Flush:17: z_axis_top:1 ↔ rope_mount_b:1
- Mate:532: rope_mount_a:1 ↔ rope_mount_holder:1
- Mate:533: rope_mount_b:1 ↔ rope_mount_holder:1
- Mate:534: rope_mount_b:1 ↔ rope_mount_holder:1
- Mate:539: z_axis_top:2 ↔ rope_mount_b:2